# Autodesk Inventor assembly: ax4_holder_asm
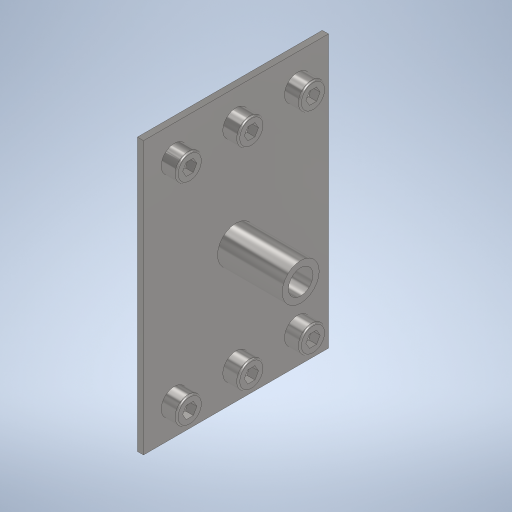
[picture p0: Inventor's stored thumbnail of the model, 512x512]
Saved by Autodesk Inventor 2024 (Build 280153000, 153)
## iProperties
Created: 2025-12-19
Part Number: ax4_holder_asm
Document SubType Name: Assembly
Designer: schar
Author: schar
## Documents named in this file (4)
- C:\Users\schar\Desktop\projectBlueprint\AMSTS\hardware\ax4_holder_asm.iam
- C:\Users\schar\Desktop\projectBlueprint\AMSTS\hardware\ax4_holder.ipt
- C:\Users\schar\Documents\Inventor\Content Center Files\R2024\en-US\ISO 4762(1)\DIN EN ISO 4762 - M5 x 8.ipt
- C:\Users\schar\Desktop\projectBlueprint\AMSTS\hardware\tnut_m5_2020.ipt
## Components (13 placed, 3 different names)
1. ax4_holder:1 — Mate:1, Mate:2, Mate:3, Mate:4, Mate:5, Mate:6, Mate:7, Mate:8, Mate:9, Mate:10, Mate:11, Mate:12, Rotational:1, Rotational:2, Rotational:3, Rotational:4, Rotational:5, Rotational:6, Mate:13, Flush:1, Flush:2
2. DIN EN ISO 4762 M5 x 8:1 — Mate:4, Mate:7
3. DIN EN ISO 4762 M5 x 8:2 — Mate:5, Mate:8
4. DIN EN ISO 4762 M5 x 8:3 — Mate:6, Mate:9
5. DIN EN ISO 4762 M5 x 8:4 — Mate:3, Mate:12
6. DIN EN ISO 4762 M5 x 8:5 — Mate:2, Mate:11
7. DIN EN ISO 4762 M5 x 8:6 — Mate:1, Mate:10
8. tnut_m5_2020:1 — Rotational:6
9. tnut_m5_2020:2 — Rotational:5
10. tnut_m5_2020:3 — Rotational:4
11. tnut_m5_2020:4 — Rotational:1
12. tnut_m5_2020:5 — Rotational:2
13. tnut_m5_2020:6 — Rotational:3
## Relationships (21: Mate 13, RevoluteJoint 6, Flush 2)
- Mate:1: ax4_holder:1 ↔ DIN EN ISO 4762 M5 x 8:6
- Mate:2: ax4_holder:1 ↔ DIN EN ISO 4762 M5 x 8:5
- Mate:3: ax4_holder:1 ↔ DIN EN ISO 4762 M5 x 8:4
- Mate:4: ax4_holder:1 ↔ DIN EN ISO 4762 M5 x 8:1
- Mate:5: ax4_holder:1 ↔ DIN EN ISO 4762 M5 x 8:2
- Mate:6: ax4_holder:1 ↔ DIN EN ISO 4762 M5 x 8:3
- Mate:7: ax4_holder:1 ↔ DIN EN ISO 4762 M5 x 8:1
- Mate:8: ax4_holder:1 ↔ DIN EN ISO 4762 M5 x 8:2
- Mate:9: ax4_holder:1 ↔ DIN EN ISO 4762 M5 x 8:3
- Mate:10: ax4_holder:1 ↔ DIN EN ISO 4762 M5 x 8:6
- Mate:11: ax4_holder:1 ↔ DIN EN ISO 4762 M5 x 8:5
- Mate:12: ax4_holder:1 ↔ DIN EN ISO 4762 M5 x 8:4
- Rotational:1 [RevoluteJoint] (0.159 mm): ax4_holder:1 ↔ tnut_m5_2020:4
- Rotational:2 [RevoluteJoint] (0.159 mm): ax4_holder:1 ↔ tnut_m5_2020:5
- Rotational:3 [RevoluteJoint] (0.159 mm): ax4_holder:1 ↔ tnut_m5_2020:6
- Rotational:4 [RevoluteJoint] (0.159 mm): ax4_holder:1 ↔ tnut_m5_2020:3
- Rotational:5 [RevoluteJoint] (0.159 mm): ax4_holder:1 ↔ tnut_m5_2020:2
- Rotational:6 [RevoluteJoint] (0.159 mm): ax4_holder:1 ↔ tnut_m5_2020:1
- Mate:13: ax4_holder:1
- Flush:1: ax4_holder:1
- Flush:2: ax4_holder:1
